# Autodesk Inventor assembly: launching unit
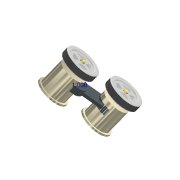
[picture p0: Inventor's stored thumbnail of the model, 180x180]
Saved by Autodesk Inventor 2021 (Build 250183000, 183)
## iProperties
Created: 2021-07-11
Part Number: launching unit
Document SubType Name: Assembly
Designer: user
Author: user
## Documents named in this file (4)
- C:\Users\user\Desktop\New folder\launching unit.iam
- C:\Users\user\Desktop\New folder\dc motor holder 2.ipt
- C:\Users\user\Desktop\New folder\cock wheel.ipt
- C:\Users\user\Desktop\New folder\dc motor 2.ipt
## Components (5 placed, 3 different names)
1. dc motor holder 2:1 — Mate:1, Mate:2, Flush:1, Flush:2
2. cock wheel:1 — Mate:4, Flush:4
3. cock wheel:2 — Mate:3, Flush:3
4. dc motor 2:1 — Mate:2, Flush:2, Mate:4, Flush:4
5. dc motor 2:2 — Mate:1, Flush:1, Mate:3, Flush:3
## Relationships (8: Mate 4, Flush 4)
- Mate:1: dc motor holder 2:1 ↔ dc motor 2:2
- Mate:2: dc motor holder 2:1 ↔ dc motor 2:1
- Flush:1 (-20 mm): dc motor holder 2:1 ↔ dc motor 2:2
- Flush:2 (-20 mm): dc motor holder 2:1 ↔ dc motor 2:1
- Mate:3: cock wheel:2 ↔ dc motor 2:2
- Mate:4: cock wheel:1 ↔ dc motor 2:1
- Flush:3 (-5 mm): cock wheel:2 ↔ dc motor 2:2
- Flush:4 (-5 mm): cock wheel:1 ↔ dc motor 2:1
